# Autodesk Inventor assembly: Kerbal Kontroller v.1
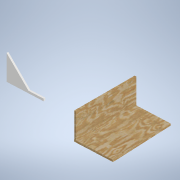
[picture p0: Inventor's stored thumbnail of the model, 180x180]
Saved by Autodesk Inventor 2021 (Build 250183000, 183)
## iProperties
Created: 2020-07-15
Part Number: Kerbal Kontroller v.1
Document SubType Name: Assembly
Designer: adick
Author: adick
## Documents named in this file (4)
- C:\Users\adick\Documents\Inventor CAD\Kerbal Kontroller v.1.iam
- C:\Users\adick\Documents\Inventor CAD\Part1.ipt
- C:\Users\adick\Documents\Inventor CAD\Part2.ipt
- C:\Users\adick\Documents\Inventor CAD\Part3.ipt
## Components (3 placed, 3 different names)
1. Part1:1 — Flush:1
2. Part2:1 — Flush:1
3. Part3:3
## Relationships (1: Flush 1)
- Flush:1: Part1:1 ↔ Part2:1
